# Autodesk Inventor assembly: frEonV2-OP3t
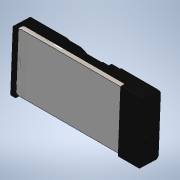
[picture p0: Inventor's stored thumbnail of the model, 180x180]
Saved by Autodesk Inventor 2020 (Build 240168000, 168)
## iProperties
Created: 2021-07-02
Part Number: frEonV2-OP3t
Document SubType Name: Assembly
Designer: dkiiv
Author: dkiiv
## Documents named in this file (4)
- D:\CAD\leeco-freon\V2\frEonV2-OP3t.iam
- D:\CAD\leeco-freon\V2\printed parts\leftOP3t.ipt
- D:\CAD\leeco-freon\V2\OnePlus3Tproper.ipt
- D:\CAD\leeco-freon\V2\right-noEONpcb-01.ipt
## Components (3 placed, 3 different names)
1. leftOP3t:1 — Mate:1, Mate:2, Mate:3
2. OnePlus3Tproper:1 — Mate:1, Mate:2, Mate:3, Mate:4, Mate:5, Mate:6
3. right-noEONpcb-01:1 — Mate:4, Mate:5, Mate:6
## Relationships (6: Mate 6)
- Mate:1: leftOP3t:1 ↔ OnePlus3Tproper:1
- Mate:2: leftOP3t:1 ↔ OnePlus3Tproper:1
- Mate:3: leftOP3t:1 ↔ OnePlus3Tproper:1
- Mate:4: OnePlus3Tproper:1 ↔ right-noEONpcb-01:1
- Mate:5: OnePlus3Tproper:1 ↔ right-noEONpcb-01:1
- Mate:6: OnePlus3Tproper:1 ↔ right-noEONpcb-01:1
